# Autodesk Inventor assembly: TigerBug
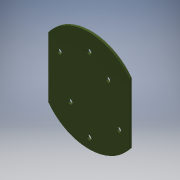
[picture p0: Inventor's stored thumbnail of the model, 180x180]
Saved by Autodesk Inventor 2016 (Build 200138000, 138)
## iProperties
Created: 2016-09-24
Part Number: TigerBug
Document SubType Name: Assembly
Designer: benja
Author: benja
## Documents named in this file (12)
- C:\Users\Ben Parnas\Google Drive\RIT FIRST club\TigerBug_\CAD\TigerBug.iam
- C:\Users\Ben Parnas\Google Drive\RIT FIRST club\TigerBug_\CAD\J024 GearMotor.iam
- C:\Users\Ben Parnas\Google Drive\RIT FIRST club\TigerBug_\CAD\PCB_PLACEHOLDER.ipt
- C:\Users\Ben Parnas\Google Drive\RIT FIRST club\TigerBug_\CAD\motorBracket_R.ipt
- C:\Users\Ben Parnas\Google Drive\RIT FIRST club\TigerBug_\CAD\adafruit 500mAh battery.ipt
- C:\Users\Ben Parnas\Google Drive\RIT FIRST club\TigerBug_\CAD\top_cover.ipt
- C:\Users\Ben Parnas\Google Drive\RIT FIRST club\TigerBug_\CAD\wheelBracket.ipt
- C:\Users\Ben Parnas\Google Drive\RIT FIRST club\TigerBug_\CAD\bumper_combined.ipt
- C:\Users\Ben Parnas\Google Drive\RIT FIRST club\TigerBug_\CAD\acorn nut94000A330_18-8 SS CAP NUT.ipt
- C:\Users\Ben Parnas\Google Drive\RIT FIRST club\TigerBug_\CAD\spacer.ipt
- C:\Users\Ben Parnas\Google Drive\RIT FIRST club\TigerBug_\CAD\KEEPOUT_TOP_0MM.ipt
- C:\Users\Ben Parnas\Google Drive\RIT FIRST club\TigerBug_\CAD\KEEPOUT_BOTTOM.ipt
## Components (17 placed, 11 different names)
1. PCB_PLACEHOLDER:1 — Mate:2, Mate:15, Mate:16, Mate:17, Mate:18, Mate:19, Mate:20, Mate:21, Mate:27, Mate:28, Mate:29, Mate:30, Mate:31, Mate:32, Mate:33, Mate:35, Flush:4, Flush:5, Mate:42, Mate:43, Mate:44, Mate:45, Flush:6, Flush:7, Flush:8, Flush:9, Flush:10, Flush:12, Flush:13, Flush:14, Flush:15, Flush:16
2. J024 GearMotor:2 [sub-assembly] — Mate:9, Mate:22, Mate:23, Mate:26
3. adafruit 500mAh battery:1 — Mate:30
4. motorBracket_R:3 — Mate:15, Mate:16, Mate:17, Mate:18, Mate:24, Mate:25
5. motorBracket_R:4 — Mate:19, Mate:20, Mate:21, Mate:22, Mate:23
6. J024 GearMotor:3 [sub-assembly] — Mate:24, Mate:25, Mate:26, Tangent:1
7. wheelBracket:1 — Mate:27, Mate:28, Mate:29, Mate:39, Mate:40, Mate:41, Angle:1
8. wheelBracket:2 — Mate:31, Mate:32, Mate:33, Mate:34, Mate:36, Mate:37, Mate:38
9. top_cover:2 — Mate:34, Mate:35
10. bumper_combined:1 — Mate:36, Mate:37, Mate:38
11. bumper_combined:2 — Mate:39, Mate:40, Mate:41, Flush:11
12. acorn nut94000A330_18-8 SS CAP NUT:1 — Insert:1
13. acorn nut94000A330_18-8 SS CAP NUT:2 — Insert:2
14. spacer:1 — Flush:4, Flush:5, Mate:42, Mate:43, Insert:1
15. spacer:2 — Mate:44, Mate:45, Insert:2
16. KEEPOUT_TOP:1 — Flush:6, Flush:7, Flush:8, Flush:9
17. KEEPOUT_BOTTOM:1 — Flush:10, Flush:11, Flush:12, Flush:13, Flush:14, Flush:15, Flush:16
## Relationships (50: Mate 33, Flush 13, Insert 2, Angle 1, Tangent 1)
- Mate:2: PCB_PLACEHOLDER:1
- Mate:9: J024 GearMotor:2
- Mate:15: PCB_PLACEHOLDER:1 ↔ motorBracket_R:3
- Mate:16: PCB_PLACEHOLDER:1 ↔ motorBracket_R:3
- Mate:17: PCB_PLACEHOLDER:1 ↔ motorBracket_R:3
- Mate:18: PCB_PLACEHOLDER:1 ↔ motorBracket_R:3
- Mate:19: PCB_PLACEHOLDER:1 ↔ motorBracket_R:4
- Mate:20: PCB_PLACEHOLDER:1 ↔ motorBracket_R:4
- Mate:21: PCB_PLACEHOLDER:1 ↔ motorBracket_R:4
- Mate:22 (0.3 mm): J024 GearMotor:2 ↔ motorBracket_R:4
- Mate:23 (0.3 mm): J024 GearMotor:2 ↔ motorBracket_R:4
- Mate:24 (0.3 mm): motorBracket_R:3 ↔ J024 GearMotor:3
- Mate:25 (0.3 mm): motorBracket_R:3 ↔ J024 GearMotor:3
- Mate:26: J024 GearMotor:2 ↔ J024 GearMotor:3
- Mate:27: PCB_PLACEHOLDER:1 ↔ wheelBracket:1
- Mate:28: PCB_PLACEHOLDER:1 ↔ wheelBracket:1
- Mate:29: PCB_PLACEHOLDER:1 ↔ wheelBracket:1
- Mate:30: PCB_PLACEHOLDER:1 ↔ adafruit 500mAh battery:1
- Mate:31: PCB_PLACEHOLDER:1 ↔ wheelBracket:2
- Mate:32: PCB_PLACEHOLDER:1 ↔ wheelBracket:2
- Mate:33: PCB_PLACEHOLDER:1 ↔ wheelBracket:2
- Mate:34: wheelBracket:2 ↔ top_cover:2
- Mate:35: PCB_PLACEHOLDER:1 ↔ top_cover:2
- Mate:36: wheelBracket:2 ↔ bumper_combined:1
- Mate:37: wheelBracket:2 ↔ bumper_combined:1
- Mate:38: wheelBracket:2 ↔ bumper_combined:1
- Mate:39: wheelBracket:1 ↔ bumper_combined:2
- Mate:40: wheelBracket:1 ↔ bumper_combined:2
- Mate:41: wheelBracket:1 ↔ bumper_combined:2
- Angle:1 (0 deg): wheelBracket:1
- Tangent:1: J024 GearMotor:3
- Flush:4: PCB_PLACEHOLDER:1 ↔ spacer:1
- Flush:5: PCB_PLACEHOLDER:1 ↔ spacer:1
- Mate:42: PCB_PLACEHOLDER:1 ↔ spacer:1
- Mate:43: PCB_PLACEHOLDER:1 ↔ spacer:1
- Mate:44: PCB_PLACEHOLDER:1 ↔ spacer:2
- Mate:45: PCB_PLACEHOLDER:1 ↔ spacer:2
- Insert:1: acorn nut94000A330_18-8 SS CAP NUT:1 ↔ spacer:1
- Insert:2: acorn nut94000A330_18-8 SS CAP NUT:2 ↔ spacer:2
- Flush:6: PCB_PLACEHOLDER:1 ↔ KEEPOUT_TOP:1
- Flush:7: PCB_PLACEHOLDER:1 ↔ KEEPOUT_TOP:1
- Flush:8: PCB_PLACEHOLDER:1 ↔ KEEPOUT_TOP:1
- Flush:9: PCB_PLACEHOLDER:1 ↔ KEEPOUT_TOP:1
- Flush:10: PCB_PLACEHOLDER:1 ↔ KEEPOUT_BOTTOM:1
- Flush:11: bumper_combined:2 ↔ KEEPOUT_BOTTOM:1
- Flush:12: PCB_PLACEHOLDER:1 ↔ KEEPOUT_BOTTOM:1
- Flush:13: PCB_PLACEHOLDER:1 ↔ KEEPOUT_BOTTOM:1
- Flush:14: PCB_PLACEHOLDER:1 ↔ KEEPOUT_BOTTOM:1
- Flush:15: PCB_PLACEHOLDER:1 ↔ KEEPOUT_BOTTOM:1
- Flush:16: PCB_PLACEHOLDER:1 ↔ KEEPOUT_BOTTOM:1
